# Autodesk Inventor assembly: module_switch
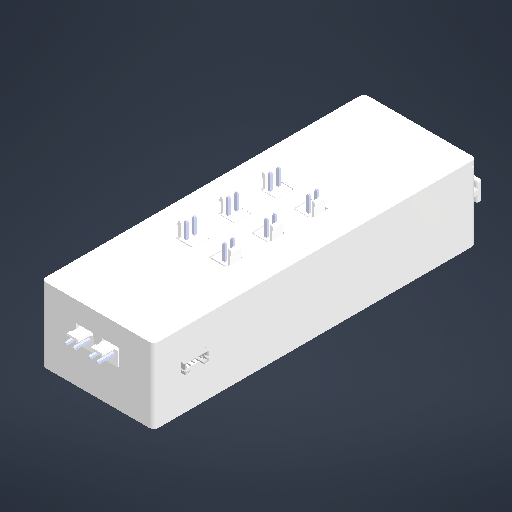
[picture p0: Inventor's stored thumbnail of the model, 512x512]
Saved by Autodesk Inventor 2025.2 (Build 292293000, 293)
## iProperties
Created: 2025-11-12
Part Number: module_switch
Document SubType Name: Assembly
Designer: sam
Author: sam
## Documents named in this file (5)
- G:\projects\primary\regulated-irrigation-system\model\asm\module-switch\module_switch.iam
- G:\projects\primary\regulated-irrigation-system\model\asm\module-switch\module_switch.ipt
- G:\projects\primary\regulated-irrigation-system\model\asm\module-switch\module-lid_switch.ipt
- G:\projects\primary\regulated-irrigation-system\model\asm\electronic-components\pcb_switch-module.iam
- G:\projects\primary\regulated-irrigation-system\model\asm\module-switch\module-switch_port-catch.ipt
## Components (4 placed, 4 different names)
1. module_switch:1 — Mate:4, Mate:5, Mate:6, Flush:1, Flush:2, Mate:7, Mate:8, Mate:9, Mate:10
2. module-lid_switch:1 — Flush:1, Flush:2, Mate:10
3. pcb_switch-module:1 [sub-assembly] — Mate:4, Mate:5, Mate:6
4. module-switch_port-catch:1 — Mate:7, Mate:8, Mate:9
## Relationships (9: Mate 7, Flush 2)
- Mate:4 (0.2 mm): module_switch:1 ↔ pcb_switch-module:1
- Mate:5: module_switch:1 ↔ pcb_switch-module:1
- Mate:6 (0.2 mm): module_switch:1 ↔ pcb_switch-module:1
- Flush:1: module_switch:1 ↔ module-lid_switch:1
- Flush:2: module_switch:1 ↔ module-lid_switch:1
- Mate:7 (0.2 mm): module_switch:1 ↔ module-switch_port-catch:1
- Mate:8 (0.2 mm): module_switch:1 ↔ module-switch_port-catch:1
- Mate:9 (0.2 mm): module_switch:1 ↔ module-switch_port-catch:1
- Mate:10: module_switch:1 ↔ module-lid_switch:1
